# Autodesk Inventor assembly: LiDAR_true
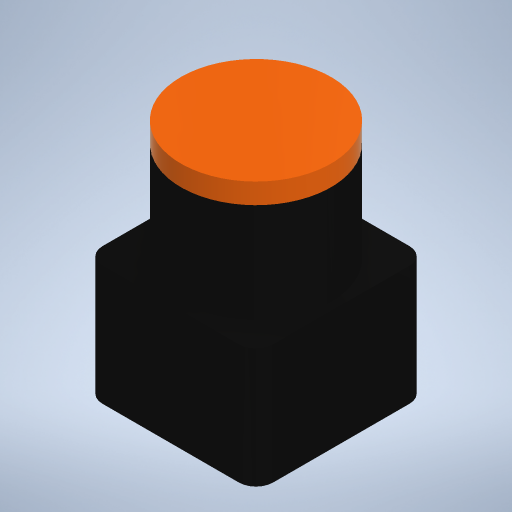
[picture p0: Inventor's stored thumbnail of the model, 512x512]
Saved by Autodesk Inventor 2023 (Build 270158000, 158)
## iProperties
Created: 2023-03-23
Part Number: LiDAR_true
Document SubType Name: Assembly
Designer: zegi
Author: zegi
## Documents named in this file (3)
- C:\Users\zegi\OneDrive - Kyushu University\2023NHK_RR_2ndvid\000_parts_zegi\sensor\LiDAR_true.iam
- C:\Users\zegi\OneDrive - Kyushu University\2023NHK_RR_2ndvid\000_parts_zegi\sensor\LiDAR_un.ipt
- C:\Users\zegi\OneDrive - Kyushu University\2023NHK_RR_2ndvid\000_parts_zegi\sensor\LiDAR_up.ipt
## Components (2 placed, 2 different names)
1. LiDAR_un:1 — 挿入:1
2. LiDAR_up:1 — 挿入:1
## Relationships (1: Insert 1)
- 挿入:1 [Insert]: LiDAR_un:1 ↔ LiDAR_up:1
